# Autodesk Inventor assembly: 6P Sprocket
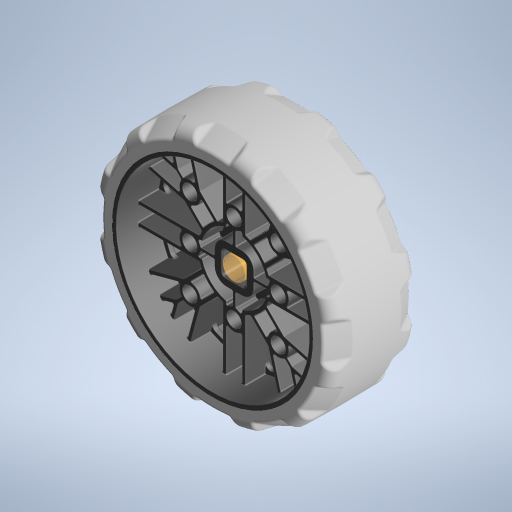
[picture p0: Inventor's stored thumbnail of the model, 512x512]
Saved by Autodesk Inventor 2023 (Build 270158000, 158)
## iProperties
Created: 2022-08-02
Part Number: 6P Sprocket
Document SubType Name: Assembly
Designer: ylu12
Author: ylu12
## Documents named in this file (3)
- C:\Users\Robodox\Documents\GitHub\2024-599Z\Cad\VEX-CAD-Inventor-1.4.0\Motion\Wheels\Traction Wheel\2.75 Traction AS, No Insert.iam
- C:\Users\Robodox\Documents\GitHub\2024-599Z\Cad\VEX-CAD-Inventor-1.4.0\Motion\Wheels\Reference Files\2.75 Traction Antistatic.ipt
- C:\Users\Robodox\Documents\GitHub\2024-599Z\Cad\VEX-CAD-Inventor-1.4.0\Motion\Wheels\Traction Wheel.iam
## Components (1 placed, 1 different names)
1. 2.75 Traction Antistatic:1 — Mate:17, Mate:18, Mate:19
## Relationships (3: Mate 3)
- Mate:17: 2.75 Traction Antistatic:1
- Mate:18: 2.75 Traction Antistatic:1
- Mate:19: 2.75 Traction Antistatic:1
## Named parameters: Thickness = 8.255 mm
